# Autodesk Inventor assembly: 付け根_1
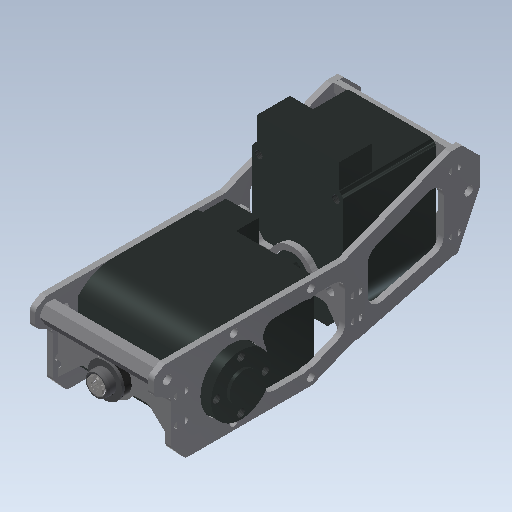
[picture p0: Inventor's stored thumbnail of the model, 512x512]
Saved by Autodesk Inventor 2020.4 (Build 244396000, 396)
## iProperties
Created: 2016-04-27
Part Number: 付け根_1
Document SubType Name: Assembly
Designer: hiroaki
Mass: 229.672 g
Surface Area: 385.784 cm^2
Volume: 116.119 cm^3
Density: 1.97789 g/cm^3
Author: hiroaki
## Documents named in this file (13)
- C:\Users\Masato\Documents\Inventor\CIT Brains_Inventor\OpenPlatform_ver3_0\下半身\足首\足首_1.iam
- C:\Users\Masato\Documents\Inventor\CIT Brains_Inventor\OpenPlatform_ver3_0\Ready_Made\B3M11xx.ipt
- C:\Users\Masato\Documents\Inventor\CIT Brains_Inventor\OpenPlatform_ver3_0\Ready_Made\free_horn.ipt
- C:\Users\Masato\Documents\Inventor\CIT Brains_Inventor\OpenPlatform_ver3_0\下半身\足首\足首_メインフレーム_1_1.ipt
- C:\Users\Masato\Documents\Inventor\CIT Brains_Inventor\OpenPlatform_ver3_0\下半身\足首\足首_サブフレーム_1_1.ipt
- C:\Users\Masato\Documents\Inventor\CIT Brains_Inventor\OpenPlatform_ver3_0\下半身\足首\足首_サブフレーム_1_2.ipt
- C:\Users\Masato\Documents\Inventor\CIT Brains_Inventor\OpenPlatform_ver3_0\下半身\足首\足首_サブフレーム_1_3.ipt
- C:\Users\Masato\Documents\Inventor\CIT Brains_Inventor\OpenPlatform_ver3_0\Ready_Made\B3M10xx.ipt
- C:\Users\Masato\Documents\Inventor\CIT Brains_Inventor\OpenPlatform_ver3_0\Ready_Made\SLSBF6-39_5-M3-N3.ipt
- C:\Users\Masato\Documents\Inventor\CIT Brains_Inventor\OpenPlatform_ver3_0\Ready_Made\BRU-307S.ipt
- C:\Users\Masato\Documents\Inventor\CIT Brains_Inventor\OpenPlatform_ver3_0\Ready_Made\S3-07-3W.ipt
- C:\Users\Masato\Documents\Inventor\CIT Brains_Inventor\OpenPlatform_ver3_0\Ready_Made\80F-0603.ipt
- C:\Users\Masato\Documents\Inventor\CIT Brains_Inventor\OpenPlatform_ver3_0\Ready_Made\CC-0612-25B.ipt
## Components (14 placed, 11 different names)
1. B3M11xx:1 — 挿入:23, 挿入:24, 挿入:25, 挿入:26, 挿入:27, 挿入:36, 挿入:51, 挿入:52, 挿入:53
2. B3M11xx:3 — 挿入:42, 挿入:43, 挿入:44, 挿入:45
3. free_horn:1 — 挿入:23
4. 足首_メインフレーム_1_1:1 — 挿入:24, 挿入:25, 挿入:26, 挿入:27, メイト:1, メイト:2, メイト:3, メイト:4, メイト:5, メイト:6, メイト:8, 挿入:54, 挿入:55
5. 足首_メインフレーム_1_1:2 — 挿入:36, 挿入:51, 挿入:52, 挿入:53, メイト:9, メイト:10
6. 足首_サブフレーム_1_1:1 — メイト:1, メイト:2, メイト:3, 挿入:42, 挿入:45
7. 足首_サブフレーム_1_2:1 — メイト:4, メイト:5, メイト:6, 挿入:43, 挿入:44
8. 足首_サブフレーム_1_3:1 — メイト:8, メイト:9, メイト:10, メイト:11, 挿入:58, 挿入:59, 挿入:60
9. SLSBF6-39_5-M3-N3:1 — 挿入:54
10. SLSBF6-39_5-M3-N3:2 — 挿入:55
11. BRU-307S:2 — 挿入:60
12. S3-07-3W:1 — メイト:11, 挿入:58
13. 80F-0603:1 — 挿入:61
14. CC-0612-25B:1 — 挿入:59, 挿入:61
## Relationships (29: Insert 19, Mate 10)
- 挿入:23 [Insert] (0.2 mm): B3M11xx:1 ↔ free_horn:1
- 挿入:24 [Insert]: B3M11xx:1 ↔ 足首_メインフレーム_1_1:1
- 挿入:25 [Insert]: B3M11xx:1 ↔ 足首_メインフレーム_1_1:1
- 挿入:26 [Insert]: B3M11xx:1 ↔ 足首_メインフレーム_1_1:1
- 挿入:27 [Insert]: B3M11xx:1 ↔ 足首_メインフレーム_1_1:1
- メイト:1 [Mate] (0.01 mm): 足首_メインフレーム_1_1:1 ↔ 足首_サブフレーム_1_1:1
- メイト:2 [Mate]: 足首_メインフレーム_1_1:1 ↔ 足首_サブフレーム_1_1:1
- メイト:3 [Mate] (0.01 mm): 足首_メインフレーム_1_1:1 ↔ 足首_サブフレーム_1_1:1
- メイト:4 [Mate]: 足首_メインフレーム_1_1:1 ↔ 足首_サブフレーム_1_2:1
- メイト:5 [Mate] (0.01 mm): 足首_メインフレーム_1_1:1 ↔ 足首_サブフレーム_1_2:1
- メイト:6 [Mate] (0.01 mm): 足首_メインフレーム_1_1:1 ↔ 足首_サブフレーム_1_2:1
- 挿入:36 [Insert]: B3M11xx:1 ↔ 足首_メインフレーム_1_1:2
- メイト:8 [Mate]: 足首_メインフレーム_1_1:1 ↔ 足首_サブフレーム_1_3:1
- 挿入:42 [Insert]: B3M11xx:3 ↔ 足首_サブフレーム_1_1:1
- 挿入:43 [Insert]: B3M11xx:3 ↔ 足首_サブフレーム_1_2:1
- 挿入:44 [Insert]: B3M11xx:3 ↔ 足首_サブフレーム_1_2:1
- 挿入:45 [Insert]: B3M11xx:3 ↔ 足首_サブフレーム_1_1:1
- 挿入:51 [Insert]: B3M11xx:1 ↔ 足首_メインフレーム_1_1:2
- 挿入:52 [Insert]: B3M11xx:1 ↔ 足首_メインフレーム_1_1:2
- 挿入:53 [Insert]: B3M11xx:1 ↔ 足首_メインフレーム_1_1:2
- メイト:9 [Mate] (0.01 mm): 足首_メインフレーム_1_1:2 ↔ 足首_サブフレーム_1_3:1
- メイト:10 [Mate] (0.01 mm): 足首_メインフレーム_1_1:2 ↔ 足首_サブフレーム_1_3:1
- 挿入:54 [Insert]: 足首_メインフレーム_1_1:1 ↔ SLSBF6-39_5-M3-N3:1
- 挿入:55 [Insert]: 足首_メインフレーム_1_1:1 ↔ SLSBF6-39_5-M3-N3:2
- メイト:11 [Mate] (0.01 mm): 足首_サブフレーム_1_3:1 ↔ S3-07-3W:1
- 挿入:58 [Insert]: 足首_サブフレーム_1_3:1 ↔ S3-07-3W:1
- 挿入:59 [Insert]: 足首_サブフレーム_1_3:1 ↔ CC-0612-25B:1
- 挿入:60 [Insert]: 足首_サブフレーム_1_3:1 ↔ BRU-307S:2
- 挿入:61 [Insert]: 80F-0603:1 ↔ CC-0612-25B:1
